# Autodesk Inventor assembly: TEMP
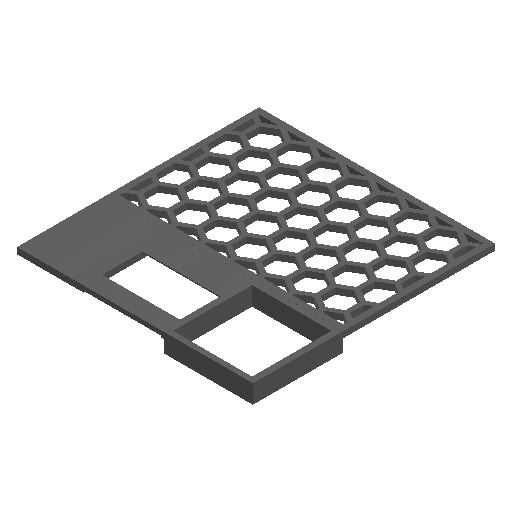
[picture p0: Inventor's stored thumbnail of the model, 512x512]
Saved by Autodesk Inventor 2026.1 (Build 301233020, 233B)
## iProperties
Created: 2026-01-15
Part Number: TEMP
Document SubType Name: Assembly
Designer: Paweł
Author: Paweł
## Documents named in this file (3)
- C:\Users\Paweł\OneDrive - Politechnika Warszawska\Dokumenty\GPS-Tracker\Models_Inventor\TEMP.iam
- C:\Users\Paweł\OneDrive - Politechnika Warszawska\Dokumenty\GPS-Tracker\Models_Inventor\pokrywka2.ipt
- C:\Users\Paweł\OneDrive - Politechnika Warszawska\Dokumenty\GPS-Tracker\Models_Inventor\honneypattern.ipt
## Components (2 placed, 2 different names)
1. pokrywka2:1 — Mate:1, Flush:1, Flush:2
2. honneypattern:1 — Mate:1, Flush:1, Flush:2
## Relationships (3: Flush 2, Mate 1)
- Mate:1: pokrywka2:1 ↔ honneypattern:1
- Flush:1: pokrywka2:1 ↔ honneypattern:1
- Flush:2: pokrywka2:1 ↔ honneypattern:1
